# Autodesk Inventor assembly: wheel 1 sprocket inner
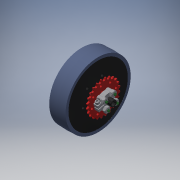
[picture p0: Inventor's stored thumbnail of the model, 180x180]
Saved by Autodesk Inventor 2018 (Build 220112000, 112)
## iProperties
Created: 2017-11-04
Part Number: wheel 1 sprocket inner
Document SubType Name: Assembly
Designer: ball
Author: ball
## Documents named in this file (13)
- C:\FTC\2017Robot\wheel 1 sprocket inner.iam
- C:\FTC\Andymark\am-2648_4inWheel8mmHub.ipt
- C:\FTC\Actobotics\545 parts\545456.ipt
- C:\FTC\Actobotics\615 parts\615106.ipt
- C:\FTC\Actobotics\545 parts\545619 assembly.ipt
- C:\FTC\Actobotics\545 parts\545619 assembly drilled out.ipt
- C:\FTC\Actobotics\545 parts\545456 counterbore.ipt
- C:\FTC\Actobotics\632 parts\632128.ipt
- C:\FTC\Actobotics\632 parts\632142.ipt
- C:\FTC\Actobotics\632 parts\632120.ipt
- C:\FTC\Actobotics\525 parts\625102 assembly.ipt
- C:\FTC\Actobotics\633 parts\633104.ipt
- C:\FTC\Actobotics\632 parts\632110.ipt
## Components (28 placed, 12 different names)
1. am-2648_4inWheel8mmHub:1 — Mate:2, Mate:3, Mate:4, Mate:11, Mate:12, Mate:13
2. 545456:1 — Mate:2, Mate:3, Mate:4, Mate:69, Mate:70, Mate:71, Mate:73, Mate:74, Mate:75, Mate:76, Mate:77, Mate:78, Mate:79
3. 615106:2 — Mate:14, Mate:15, Mate:16, Mate:21, Mate:22, Mate:23
4. 545619 assembly:1 — Mate:45, Mate:69, Mate:70, Mate:71, Mate:72
5. 545619 assembly drilled out:1 — Mate:14, Mate:15, Mate:16, Mate:24, Mate:25, Mate:26, Mate:27, Mate:28, Mate:29, Mate:30, Mate:31, Mate:55, Mate:56
6. 545456 counterbore:1 — Mate:11, Mate:12, Mate:13, Mate:17, Mate:18, Mate:21, Mate:22, Mate:23, Mate:57, Mate:58, Mate:59, Mate:60, Mate:61, Mate:62, Mate:63, Mate:64, Mate:65, Mate:66, Mate:67, Mate:68
7. 632128:1 — Mate:17, Mate:18
8. 632120:2
9. 632142:2 — Mate:24, Mate:25
10. 632142:3 — Mate:30, Mate:31
11. 632142:4 — Mate:28, Mate:29
12. 632142:5 — Mate:26, Mate:27
13. 625102 assembly:3 — Mate:45, Mate:80
14. 633104:1 — Mate:47, Mate:48, Mate:49, Mate:51, Mate:53, Mate:55, Mate:56
15. 633104:2 — Mate:47, Mate:48, Mate:50
16. 633104:3 — Mate:53, Mate:54, Mate:80
17. 633104:4 — Mate:51, Mate:52, Mate:54
18. 633104:5 — Mate:49, Mate:50, Mate:52
19. 632120:3 — Mate:61, Mate:62
20. 632120:4 — Mate:59, Mate:60
21. 632120:5 — Mate:57, Mate:58
22. 632128:2 — Mate:63, Mate:64
23. 632128:3 — Mate:65, Mate:66
24. 632128:4 — Mate:67, Mate:68
25. 632110:1 — Mate:72, Mate:75
26. 632110:2 — Mate:76, Mate:77
27. 632110:3 — Mate:78, Mate:79
28. 632110:4 — Mate:73, Mate:74
## Relationships (59: Mate 59)
- Mate:2: am-2648_4inWheel8mmHub:1 ↔ 545456:1
- Mate:3: am-2648_4inWheel8mmHub:1 ↔ 545456:1
- Mate:4: am-2648_4inWheel8mmHub:1 ↔ 545456:1
- Mate:11: am-2648_4inWheel8mmHub:1 ↔ 545456 counterbore:1
- Mate:12: am-2648_4inWheel8mmHub:1 ↔ 545456 counterbore:1
- Mate:13: am-2648_4inWheel8mmHub:1 ↔ 545456 counterbore:1
- Mate:14: 615106:2 ↔ 545619 assembly drilled out:1
- Mate:15: 615106:2 ↔ 545619 assembly drilled out:1
- Mate:16: 615106:2 ↔ 545619 assembly drilled out:1
- Mate:17: 545456 counterbore:1 ↔ 632128:1
- Mate:18: 545456 counterbore:1 ↔ 632128:1
- [Mate]: 545456 counterbore:1 ↔ 632120:2
- [Mate]: 545456 counterbore:1 ↔ 632120:2
- Mate:21: 615106:2 ↔ 545456 counterbore:1
- Mate:22: 615106:2 ↔ 545456 counterbore:1
- Mate:23: 615106:2 ↔ 545456 counterbore:1
- Mate:24: 545619 assembly drilled out:1 ↔ 632142:2
- Mate:25: 545619 assembly drilled out:1 ↔ 632142:2
- Mate:26: 545619 assembly drilled out:1 ↔ 632142:5
- Mate:27: 545619 assembly drilled out:1 ↔ 632142:5
- Mate:28: 545619 assembly drilled out:1 ↔ 632142:4
- Mate:29: 545619 assembly drilled out:1 ↔ 632142:4
- Mate:30: 545619 assembly drilled out:1 ↔ 632142:3
- Mate:31: 545619 assembly drilled out:1 ↔ 632142:3
- Mate:45: 545619 assembly:1 ↔ 625102 assembly:3
- Mate:47: 633104:1 ↔ 633104:2
- Mate:48: 633104:1 ↔ 633104:2
- Mate:49: 633104:1 ↔ 633104:5
- Mate:50: 633104:2 ↔ 633104:5
- Mate:51: 633104:1 ↔ 633104:4
- Mate:52: 633104:4 ↔ 633104:5
- Mate:53: 633104:1 ↔ 633104:3
- Mate:54: 633104:3 ↔ 633104:4
- Mate:55: 545619 assembly drilled out:1 ↔ 633104:1
- Mate:56: 545619 assembly drilled out:1 ↔ 633104:1
- Mate:57: 545456 counterbore:1 ↔ 632120:5
- Mate:58: 545456 counterbore:1 ↔ 632120:5
- Mate:59: 545456 counterbore:1 ↔ 632120:4
- Mate:60: 545456 counterbore:1 ↔ 632120:4
- Mate:61: 545456 counterbore:1 ↔ 632120:3
- Mate:62: 545456 counterbore:1 ↔ 632120:3
- Mate:63: 545456 counterbore:1 ↔ 632128:2
- Mate:64: 545456 counterbore:1 ↔ 632128:2
- Mate:65: 545456 counterbore:1 ↔ 632128:3
- Mate:66: 545456 counterbore:1 ↔ 632128:3
- Mate:67: 545456 counterbore:1 ↔ 632128:4
- Mate:68: 545456 counterbore:1 ↔ 632128:4
- Mate:69: 545456:1 ↔ 545619 assembly:1
- Mate:70: 545456:1 ↔ 545619 assembly:1
- Mate:71: 545456:1 ↔ 545619 assembly:1
- Mate:72: 545619 assembly:1 ↔ 632110:1
- Mate:73: 545456:1 ↔ 632110:4
- Mate:74: 545456:1 ↔ 632110:4
- Mate:75: 545456:1 ↔ 632110:1
- Mate:76: 545456:1 ↔ 632110:2
- Mate:77: 545456:1 ↔ 632110:2
- Mate:78: 545456:1 ↔ 632110:3
- Mate:79: 545456:1 ↔ 632110:3
- Mate:80 (-73.406 mm): 625102 assembly:3 ↔ 633104:3
